# Autodesk Inventor assembly: GP4-100
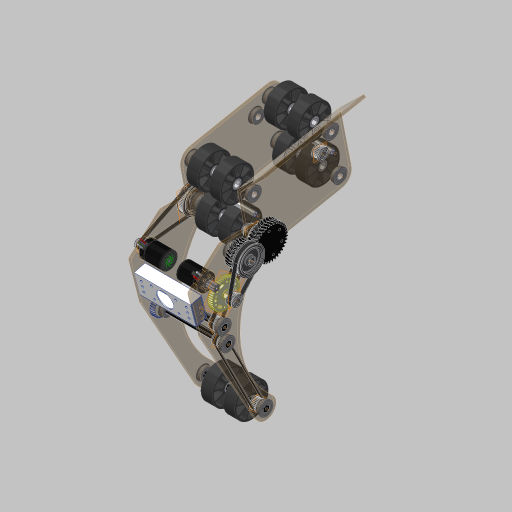
[picture p0: Inventor's stored thumbnail of the model, 512x512]
Saved by Autodesk Inventor 2023.5 (Build 275446000, 446)
## iProperties
Created: 2025-01-28
Part Number: GP4-100
Document SubType Name: Assembly
Designer: slick
Mass: 3583.72 g
Surface Area: 9499.92 cm^2
Volume: 1982.36 cm^3
Density: 1.80781 g/cm^3
Author: slick
## Documents named in this file (26)
- C:\Users\slick\OneDrive\Desktop\2025-ReefScape---CAD\Gripper\GP4\GP4-100.iam
- C:\Users\slick\OneDrive\Desktop\2025-ReefScape---CAD\Gripper\GP4\GP4-001.ipt
- C:\Users\slick\OneDrive\Desktop\2025-ReefScape---CAD\Gripper\GP4\GP4-002.ipt
- C:\Users\slick\OneDrive\Desktop\2025-ReefScape---CAD\Gripper\GP4\GP4-003.ipt
- C:\Users\slick\OneDrive\Desktop\2025-ReefScape---CAD\Gripper\GP4\GP4-003_MIR.ipt
- C:\Users\slick\OneDrive\Desktop\2025-ReefScape---CAD\COMMON PARTS\WHEELS\am-3945 3IN 500Hex Compliant Wheel REV 3.ipt
- C:\Users\slick\OneDrive\Desktop\2025-ReefScape---CAD\Gripper\GP4\GP4-005.ipt
- C:\Users\slick\OneDrive\Desktop\2025-ReefScape---CAD\Gripper\GP4\GP4-006.ipt
- C:\Users\slick\OneDrive\Desktop\2025-ReefScape---CAD\Gripper\GP4\GP4-007.ipt
- C:\Users\slick\OneDrive\Desktop\2025-ReefScape---CAD\COMMON PARTS\MOTORS\Minion.ipt
- C:\Users\slick\OneDrive\Desktop\2025-ReefScape---CAD\COMMON PARTS\PULLEYS\gt2\16T Gt2 Kracken PullyWCP-1178.ipt
- C:\Users\slick\OneDrive\Desktop\2025-ReefScape---CAD\COMMON PARTS\BEARINGS\13_75mm_1_2_ThunderHex_ID_x_1_125_OD_x_0_313_WD_Flanged_Bearing_217-4006_MIR.ipt
- C:\Users\slick\OneDrive\Desktop\2025-ReefScape---CAD\Gripper\GP4\GP4-008.ipt
- C:\Users\slick\OneDrive\Desktop\2025-ReefScape---CAD\COMMON PARTS\PULLEYS\gt2\60t_x_9mm_Wide_Double_Flange_Aluminum_Pulley_GT2_3mm_1_2_Hex_Bore_217-5876.ipt
- C:\Users\slick\OneDrive\Desktop\2025-ReefScape---CAD\COMMON PARTS\PULLEYS\gt2\24t_x_9mm_Wide_Double_Flange_Aluminum_Pulley_GT2_3mm_1_2_Hex_Bore_217-5875.ipt
- C:\Users\slick\OneDrive\Desktop\2025-ReefScape---CAD\COMMON PARTS\GEARS\20dp .5 hex\30t_Aluminum_Spur_Gear_20_DP_1_2_Hex_Bore_217-2705.ipt
- C:\Users\slick\OneDrive\Desktop\2025-ReefScape---CAD\Gripper\GP4\GP4-009.ipt
- C:\Users\slick\OneDrive\Desktop\2025-ReefScape---CAD\Gripper\GP4\GP4-010.ipt
- C:\Users\slick\OneDrive\Desktop\2025-ReefScape---CAD\COMMON PARTS\GEARS\Herringbone\herringbone 2m 24t\herringbone 2m 24t.ipt
- C:\Users\slick\OneDrive\Desktop\2025-ReefScape---CAD\COMMON PARTS\GEARS\Herringbone\2m 36t herringbone\2m 36t herringbone.ipt
- C:\Users\slick\OneDrive\Desktop\2025-ReefScape---CAD\COMMON PARTS\GEARS\WCP-1006\WCP-1006.ipt
- C:\Users\slick\OneDrive\Desktop\2025-ReefScape---CAD\COMMON PARTS\GEARS\20dp .5 hex\48t_Aluminum_Spur_Gear_20_DP_1_2_Hex_Bore_VersaKeys_217-3218.ipt
- C:\Users\slick\OneDrive\Desktop\2025-ReefScape---CAD\Gripper\GP4\90T GT2 Belt.ipt
- C:\Users\slick\OneDrive\Desktop\2025-ReefScape---CAD\Gripper\GP4\150T GT2 Belt.ipt
- C:\Users\slick\OneDrive\Desktop\2025-ReefScape---CAD\Gripper\GP4\130T GT2 Belt.ipt
- C:\Users\slick\OneDrive\Desktop\2025-ReefScape---CAD\Gripper\GP4\120T GT2 Belt.ipt
## Components (63 placed, 25 different names)
1. GP4-008:1 — Insert:1, Insert:2, Mate:2, Mate:6, Mate:11, Insert:21, Insert:26, Insert:27, Insert:28, Mate:41, Mate:42, Insert:29, Insert:30, Mate:49
2. GP4-002:1 — Flush:1, Flush:2, Flush:3, Mate:1, Flush:4, Flush:5
3. GP4-003:1 — Flush:1, Mate:1, Flush:4, Insert:1, Insert:2
4. GP4-003_MIR:1 — Flush:2, Flush:3, Flush:5, Insert:3, Insert:4
5. GP4-001:2 — Insert:3, Insert:4, Mate:7, Mate:10, Mate:12, Mate:23, Mate:24, Insert:7, Insert:14, Insert:15, Insert:16, Mate:27, Insert:19
6. GP4-006:1 — Mate:12, Mate:20, Mate:21, Mate:22, Symmetry:1, Insert:11, Insert:12, Insert:13, Mate:27, Insert:17, Insert:18, Insert:20, Insert:32, Mate:55
7. GP4-005:2 — Mate:11, Mate:15, Mate:22, Symmetry:1, Insert:5, Insert:6, Insert:22, Insert:23, Insert:24, Insert:25, Insert:33, Insert:34
8. GP4-007:1 — Insert:6, Insert:18
9. GP4-007:2 — Insert:5, Insert:17
10. Minion:1 — Mate:23, Mate:24, Insert:7, Mate:25, Flush:11, Mate:63
11. 16T Gt2 Kracken PullyWCP-1178:1 — Mate:25, Flush:11, Flush:29, Flush:30
12. 60t_x_9mm_Wide_Double_Flange_Aluminum_Pulley_GT2_3mm_1_2_Hex_Bore_217-5876:1 — Mate:28, Mate:54, Mate:61, Mate:64, Flush:30
13. 24t_x_9mm_Wide_Double_Flange_Aluminum_Pulley_GT2_3mm_1_2_Hex_Bore_217-5875:1 — Mate:32, Flush:14
14. 24t_x_9mm_Wide_Double_Flange_Aluminum_Pulley_GT2_3mm_1_2_Hex_Bore_217-5875:2 — Mate:31, Flush:13, Flush:14, Mate:62
15. 24t_x_9mm_Wide_Double_Flange_Aluminum_Pulley_GT2_3mm_1_2_Hex_Bore_217-5875:3 — Mate:30, Flush:13, Flush:17
16. 24t_x_9mm_Wide_Double_Flange_Aluminum_Pulley_GT2_3mm_1_2_Hex_Bore_217-5875:4 — Mate:29, Mate:37, Flush:17, Flush:28
17. 30t_Aluminum_Spur_Gear_20_DP_1_2_Hex_Bore_217-2705:1 — Mate:34, Flush:16, Mate:36, Mate:39, Flush:19
18. 30t_Aluminum_Spur_Gear_20_DP_1_2_Hex_Bore_217-2705:2 — Mate:35, Flush:16, Mate:38, Flush:18
19. GP4-009:1 — Mate:38, Flush:18
20. GP4-009:2 — Mate:39, Flush:19
21. GP4-010:1 — Mate:40, Flush:20
22. Minion:2 — Mate:41, Mate:42, Insert:29, Mate:48, Flush:23
23. herringbone 2m 24t:1 — Mate:44, Flush:22, Rotation:1, Mate:51, Mate:53
24. 24t_x_9mm_Wide_Double_Flange_Aluminum_Pulley_GT2_3mm_1_2_Hex_Bore_217-5875:5 — Mate:46, Flush:25
25. 24t_x_9mm_Wide_Double_Flange_Aluminum_Pulley_GT2_3mm_1_2_Hex_Bore_217-5875:6 — Mate:47
26. 2m 36t herringbone:1 — Insert:33, Insert:34, Flush:22, Rotation:1
27. WCP-1006:1 — Mate:48, Flush:23, Flush:26
28. 48t_Aluminum_Spur_Gear_20_DP_1_2_Hex_Bore_VersaKeys_217-3218:1 — Mate:49, Mate:50, Flush:26
29. 60t_x_9mm_Wide_Double_Flange_Aluminum_Pulley_GT2_3mm_1_2_Hex_Bore_217-5876:2 — Mate:51, Mate:53, Flush:24, Mate:57
30. 24t_x_9mm_Wide_Double_Flange_Aluminum_Pulley_GT2_3mm_1_2_Hex_Bore_217-5875:7 — Mate:50, Flush:24, Mate:56, Flush:27
31. 24t_x_9mm_Wide_Double_Flange_Aluminum_Pulley_GT2_3mm_1_2_Hex_Bore_217-5875:8 — Mate:54, Flush:25, Mate:55
32. 90T GT2 Belt:1 — Mate:56, Mate:57, Flush:27
33. 150T GT2 Belt:1 — Mate:58, Mate:59, Flush:28
34. 130T GT2 Belt:1 — Mate:60, Mate:61, Mate:62
35. 120T GT2 Belt:1 — Mate:63, Mate:64, Flush:29
36. am-3945 3IN 500Hex Compliant Wheel REV 3:10
37. am-3945 3IN 500Hex Compliant Wheel REV 3:9 — Mate:21, Flush:9
38. am-3945 3IN 500Hex Compliant Wheel REV 3:8
39. am-3945 3IN 500Hex Compliant Wheel REV 3:7 — Mate:20, Flush:10
40. am-3945 3IN 500Hex Compliant Wheel REV 3:6 — Mate:2, Mate:3, Flush:6, Flush:9
41. am-3945 3IN 500Hex Compliant Wheel REV 3:5 — Mate:3, Flush:7, Mate:10
42. am-3945 3IN 500Hex Compliant Wheel REV 3:4 — Mate:6, Mate:8
43. am-3945 3IN 500Hex Compliant Wheel REV 3:3 — Mate:7, Mate:8, Flush:8
44. am-3945 3IN 500Hex Compliant Wheel REV 3:2 — Mate:5, Mate:9, Flush:7, Flush:8
45. am-3945 3IN 500Hex Compliant Wheel REV 3:1 — Mate:5, Mate:9, Flush:6, Mate:15, Flush:10
46. 13_75mm_1_2_ThunderHex_ID_x_1_125_OD_x_0_313_WD_Flanged_Bearing_217-4006_MIR:19 — Insert:32, Mate:47
47. 13_75mm_1_2_ThunderHex_ID_x_1_125_OD_x_0_313_WD_Flanged_Bearing_217-4006_MIR:18 — Insert:30, Mate:44
48. 13_75mm_1_2_ThunderHex_ID_x_1_125_OD_x_0_313_WD_Flanged_Bearing_217-4006_MIR:10 — Insert:21
49. 13_75mm_1_2_ThunderHex_ID_x_1_125_OD_x_0_313_WD_Flanged_Bearing_217-4006_MIR:11 — Insert:22
50. 13_75mm_1_2_ThunderHex_ID_x_1_125_OD_x_0_313_WD_Flanged_Bearing_217-4006_MIR:12 — Insert:23
51. 13_75mm_1_2_ThunderHex_ID_x_1_125_OD_x_0_313_WD_Flanged_Bearing_217-4006_MIR:13 — Insert:24
52. 13_75mm_1_2_ThunderHex_ID_x_1_125_OD_x_0_313_WD_Flanged_Bearing_217-4006_MIR:14 — Insert:25
53. 13_75mm_1_2_ThunderHex_ID_x_1_125_OD_x_0_313_WD_Flanged_Bearing_217-4006_MIR:15 — Insert:28, Mate:60
54. 13_75mm_1_2_ThunderHex_ID_x_1_125_OD_x_0_313_WD_Flanged_Bearing_217-4006_MIR:16 — Insert:27, Mate:59
55. 13_75mm_1_2_ThunderHex_ID_x_1_125_OD_x_0_313_WD_Flanged_Bearing_217-4006_MIR:17 — Insert:26, Mate:37, Mate:58
56. 13_75mm_1_2_ThunderHex_ID_x_1_125_OD_x_0_313_WD_Flanged_Bearing_217-4006_MIR:1 — Insert:15, Mate:30, Mate:35
57. 13_75mm_1_2_ThunderHex_ID_x_1_125_OD_x_0_313_WD_Flanged_Bearing_217-4006_MIR:3 — Insert:20, Mate:32
58. 13_75mm_1_2_ThunderHex_ID_x_1_125_OD_x_0_313_WD_Flanged_Bearing_217-4006_MIR:4 — Insert:14, Mate:31, Mate:34, Mate:36
59. 13_75mm_1_2_ThunderHex_ID_x_1_125_OD_x_0_313_WD_Flanged_Bearing_217-4006_MIR:5 — Insert:13
60. 13_75mm_1_2_ThunderHex_ID_x_1_125_OD_x_0_313_WD_Flanged_Bearing_217-4006_MIR:6 — Insert:12
61. 13_75mm_1_2_ThunderHex_ID_x_1_125_OD_x_0_313_WD_Flanged_Bearing_217-4006_MIR:7 — Insert:11, Mate:46
62. 13_75mm_1_2_ThunderHex_ID_x_1_125_OD_x_0_313_WD_Flanged_Bearing_217-4006_MIR:8 — Insert:19, Mate:28
63. 13_75mm_1_2_ThunderHex_ID_x_1_125_OD_x_0_313_WD_Flanged_Bearing_217-4006_MIR:9 — Insert:16, Mate:29, Mate:40, Flush:20
## Relationships (115: Mate 56, Insert 30, Flush 27, Symmetry 1, RelateRotation 1)
- Flush:1: GP4-002:1 ↔ GP4-003:1
- Flush:2: GP4-002:1 ↔ GP4-003_MIR:1
- Flush:3: GP4-002:1 ↔ GP4-003_MIR:1
- Mate:1: GP4-002:1 ↔ GP4-003:1
- Flush:4: GP4-002:1 ↔ GP4-003:1
- Flush:5: GP4-002:1 ↔ GP4-003_MIR:1
- Insert:1: GP4-008:1 ↔ GP4-003:1
- Insert:2: GP4-008:1 ↔ GP4-003:1
- Insert:3: GP4-003_MIR:1 ↔ GP4-001:2
- Insert:4: GP4-003_MIR:1 ↔ GP4-001:2
- Mate:2: GP4-008:1 ↔ am-3945 3IN 500Hex Compliant Wheel REV 3:6
- Mate:3: am-3945 3IN 500Hex Compliant Wheel REV 3:6 ↔ am-3945 3IN 500Hex Compliant Wheel REV 3:5
- Mate:5: am-3945 3IN 500Hex Compliant Wheel REV 3:2 ↔ am-3945 3IN 500Hex Compliant Wheel REV 3:1
- Mate:6: GP4-008:1 ↔ am-3945 3IN 500Hex Compliant Wheel REV 3:4
- Mate:7: GP4-001:2 ↔ am-3945 3IN 500Hex Compliant Wheel REV 3:3
- Mate:8 (25.4 mm): am-3945 3IN 500Hex Compliant Wheel REV 3:4 ↔ am-3945 3IN 500Hex Compliant Wheel REV 3:3
- Mate:9 (25.4 mm): am-3945 3IN 500Hex Compliant Wheel REV 3:2 ↔ am-3945 3IN 500Hex Compliant Wheel REV 3:1
- Flush:6: am-3945 3IN 500Hex Compliant Wheel REV 3:6 ↔ am-3945 3IN 500Hex Compliant Wheel REV 3:1
- Flush:7: am-3945 3IN 500Hex Compliant Wheel REV 3:5 ↔ am-3945 3IN 500Hex Compliant Wheel REV 3:2
- Mate:10 (25.4 mm): GP4-001:2 ↔ am-3945 3IN 500Hex Compliant Wheel REV 3:5
- Flush:8: am-3945 3IN 500Hex Compliant Wheel REV 3:3 ↔ am-3945 3IN 500Hex Compliant Wheel REV 3:2
- Mate:11: GP4-008:1 ↔ GP4-005:2
- Mate:12: GP4-001:2 ↔ GP4-006:1
- Mate:15: GP4-005:2 ↔ am-3945 3IN 500Hex Compliant Wheel REV 3:1
- [Mate]: am-3945 3IN 500Hex Compliant Wheel REV 3:8 ↔ am-3945 3IN 500Hex Compliant Wheel REV 3:7
- [Mate] (25.4 mm): am-3945 3IN 500Hex Compliant Wheel REV 3:8 ↔ am-3945 3IN 500Hex Compliant Wheel REV 3:7
- [Mate]: am-3945 3IN 500Hex Compliant Wheel REV 3:10 ↔ am-3945 3IN 500Hex Compliant Wheel REV 3:9
- [Mate] (25.4 mm): am-3945 3IN 500Hex Compliant Wheel REV 3:10 ↔ am-3945 3IN 500Hex Compliant Wheel REV 3:9
- Mate:20: GP4-006:1 ↔ am-3945 3IN 500Hex Compliant Wheel REV 3:7
- Mate:21: GP4-006:1 ↔ am-3945 3IN 500Hex Compliant Wheel REV 3:9
- Flush:9: am-3945 3IN 500Hex Compliant Wheel REV 3:9 ↔ am-3945 3IN 500Hex Compliant Wheel REV 3:6
- Flush:10: am-3945 3IN 500Hex Compliant Wheel REV 3:7 ↔ am-3945 3IN 500Hex Compliant Wheel REV 3:1
- Mate:22: GP4-006:1 ↔ GP4-005:2
- Symmetry:1: GP4-006:1 ↔ GP4-005:2
- Insert:5: GP4-005:2 ↔ GP4-007:2
- Insert:6: GP4-005:2 ↔ GP4-007:1
- Mate:23: GP4-001:2 ↔ Minion:1
- Mate:24: GP4-001:2 ↔ Minion:1
- Insert:7: GP4-001:2 ↔ Minion:1
- Mate:25: Minion:1 ↔ 16T Gt2 Kracken PullyWCP-1178:1
- Flush:11: Minion:1 ↔ 16T Gt2 Kracken PullyWCP-1178:1
- Insert:11: GP4-006:1 ↔ 13_75mm_1_2_ThunderHex_ID_x_1_125_OD_x_0_313_WD_Flanged_Bearing_217-4006_MIR:7
- Insert:12: GP4-006:1 ↔ 13_75mm_1_2_ThunderHex_ID_x_1_125_OD_x_0_313_WD_Flanged_Bearing_217-4006_MIR:6
- Insert:13: GP4-006:1 ↔ 13_75mm_1_2_ThunderHex_ID_x_1_125_OD_x_0_313_WD_Flanged_Bearing_217-4006_MIR:5
- Insert:14: GP4-001:2 ↔ 13_75mm_1_2_ThunderHex_ID_x_1_125_OD_x_0_313_WD_Flanged_Bearing_217-4006_MIR:4
- Insert:15: GP4-001:2 ↔ 13_75mm_1_2_ThunderHex_ID_x_1_125_OD_x_0_313_WD_Flanged_Bearing_217-4006_MIR:1
- Insert:16: GP4-001:2 ↔ 13_75mm_1_2_ThunderHex_ID_x_1_125_OD_x_0_313_WD_Flanged_Bearing_217-4006_MIR:9
- Mate:27: GP4-001:2 ↔ GP4-006:1
- Insert:17: GP4-006:1 ↔ GP4-007:2
- Insert:18: GP4-006:1 ↔ GP4-007:1
- Insert:19: GP4-001:2 ↔ 13_75mm_1_2_ThunderHex_ID_x_1_125_OD_x_0_313_WD_Flanged_Bearing_217-4006_MIR:8
- Insert:20: GP4-006:1 ↔ 13_75mm_1_2_ThunderHex_ID_x_1_125_OD_x_0_313_WD_Flanged_Bearing_217-4006_MIR:3
- Mate:28: 60t_x_9mm_Wide_Double_Flange_Aluminum_Pulley_GT2_3mm_1_2_Hex_Bore_217-5876:1 ↔ 13_75mm_1_2_ThunderHex_ID_x_1_125_OD_x_0_313_WD_Flanged_Bearing_217-4006_MIR:8
- Mate:29: 24t_x_9mm_Wide_Double_Flange_Aluminum_Pulley_GT2_3mm_1_2_Hex_Bore_217-5875:4 ↔ 13_75mm_1_2_ThunderHex_ID_x_1_125_OD_x_0_313_WD_Flanged_Bearing_217-4006_MIR:9
- Mate:30: 24t_x_9mm_Wide_Double_Flange_Aluminum_Pulley_GT2_3mm_1_2_Hex_Bore_217-5875:3 ↔ 13_75mm_1_2_ThunderHex_ID_x_1_125_OD_x_0_313_WD_Flanged_Bearing_217-4006_MIR:1
- Mate:31: 24t_x_9mm_Wide_Double_Flange_Aluminum_Pulley_GT2_3mm_1_2_Hex_Bore_217-5875:2 ↔ 13_75mm_1_2_ThunderHex_ID_x_1_125_OD_x_0_313_WD_Flanged_Bearing_217-4006_MIR:4
- Mate:32: 24t_x_9mm_Wide_Double_Flange_Aluminum_Pulley_GT2_3mm_1_2_Hex_Bore_217-5875:1 ↔ 13_75mm_1_2_ThunderHex_ID_x_1_125_OD_x_0_313_WD_Flanged_Bearing_217-4006_MIR:3
- Flush:13: 24t_x_9mm_Wide_Double_Flange_Aluminum_Pulley_GT2_3mm_1_2_Hex_Bore_217-5875:2 ↔ 24t_x_9mm_Wide_Double_Flange_Aluminum_Pulley_GT2_3mm_1_2_Hex_Bore_217-5875:3
- Flush:14: 24t_x_9mm_Wide_Double_Flange_Aluminum_Pulley_GT2_3mm_1_2_Hex_Bore_217-5875:1 ↔ 24t_x_9mm_Wide_Double_Flange_Aluminum_Pulley_GT2_3mm_1_2_Hex_Bore_217-5875:2
- Mate:34: 30t_Aluminum_Spur_Gear_20_DP_1_2_Hex_Bore_217-2705:1 ↔ 13_75mm_1_2_ThunderHex_ID_x_1_125_OD_x_0_313_WD_Flanged_Bearing_217-4006_MIR:4
- Mate:35: 30t_Aluminum_Spur_Gear_20_DP_1_2_Hex_Bore_217-2705:2 ↔ 13_75mm_1_2_ThunderHex_ID_x_1_125_OD_x_0_313_WD_Flanged_Bearing_217-4006_MIR:1
- Flush:16: 30t_Aluminum_Spur_Gear_20_DP_1_2_Hex_Bore_217-2705:1 ↔ 30t_Aluminum_Spur_Gear_20_DP_1_2_Hex_Bore_217-2705:2
- Mate:36 (3.175 mm): 30t_Aluminum_Spur_Gear_20_DP_1_2_Hex_Bore_217-2705:1 ↔ 13_75mm_1_2_ThunderHex_ID_x_1_125_OD_x_0_313_WD_Flanged_Bearing_217-4006_MIR:4
- Insert:21: GP4-008:1 ↔ 13_75mm_1_2_ThunderHex_ID_x_1_125_OD_x_0_313_WD_Flanged_Bearing_217-4006_MIR:10
- Insert:22: GP4-005:2 ↔ 13_75mm_1_2_ThunderHex_ID_x_1_125_OD_x_0_313_WD_Flanged_Bearing_217-4006_MIR:11
- Insert:23: GP4-005:2 ↔ 13_75mm_1_2_ThunderHex_ID_x_1_125_OD_x_0_313_WD_Flanged_Bearing_217-4006_MIR:12
- Insert:24: GP4-005:2 ↔ 13_75mm_1_2_ThunderHex_ID_x_1_125_OD_x_0_313_WD_Flanged_Bearing_217-4006_MIR:13
- Insert:25: GP4-005:2 ↔ 13_75mm_1_2_ThunderHex_ID_x_1_125_OD_x_0_313_WD_Flanged_Bearing_217-4006_MIR:14
- Insert:26: GP4-008:1 ↔ 13_75mm_1_2_ThunderHex_ID_x_1_125_OD_x_0_313_WD_Flanged_Bearing_217-4006_MIR:17
- Insert:27: GP4-008:1 ↔ 13_75mm_1_2_ThunderHex_ID_x_1_125_OD_x_0_313_WD_Flanged_Bearing_217-4006_MIR:16
- Insert:28: GP4-008:1 ↔ 13_75mm_1_2_ThunderHex_ID_x_1_125_OD_x_0_313_WD_Flanged_Bearing_217-4006_MIR:15
- Mate:37 (3.175 mm): 24t_x_9mm_Wide_Double_Flange_Aluminum_Pulley_GT2_3mm_1_2_Hex_Bore_217-5875:4 ↔ 13_75mm_1_2_ThunderHex_ID_x_1_125_OD_x_0_313_WD_Flanged_Bearing_217-4006_MIR:17
- Flush:17: 24t_x_9mm_Wide_Double_Flange_Aluminum_Pulley_GT2_3mm_1_2_Hex_Bore_217-5875:3 ↔ 24t_x_9mm_Wide_Double_Flange_Aluminum_Pulley_GT2_3mm_1_2_Hex_Bore_217-5875:4
- Mate:38: 30t_Aluminum_Spur_Gear_20_DP_1_2_Hex_Bore_217-2705:2 ↔ GP4-009:1
- Mate:39: 30t_Aluminum_Spur_Gear_20_DP_1_2_Hex_Bore_217-2705:1 ↔ GP4-009:2
- Flush:18: 30t_Aluminum_Spur_Gear_20_DP_1_2_Hex_Bore_217-2705:2 ↔ GP4-009:1
- Flush:19: 30t_Aluminum_Spur_Gear_20_DP_1_2_Hex_Bore_217-2705:1 ↔ GP4-009:2
- Mate:40: GP4-010:1 ↔ 13_75mm_1_2_ThunderHex_ID_x_1_125_OD_x_0_313_WD_Flanged_Bearing_217-4006_MIR:9
- Flush:20: GP4-010:1 ↔ 13_75mm_1_2_ThunderHex_ID_x_1_125_OD_x_0_313_WD_Flanged_Bearing_217-4006_MIR:9
- Mate:41: GP4-008:1 ↔ Minion:2
- Mate:42: GP4-008:1 ↔ Minion:2
- Insert:29: GP4-008:1 ↔ Minion:2
- Insert:30: GP4-008:1 ↔ 13_75mm_1_2_ThunderHex_ID_x_1_125_OD_x_0_313_WD_Flanged_Bearing_217-4006_MIR:18
- Mate:44: herringbone 2m 24t:1 ↔ 13_75mm_1_2_ThunderHex_ID_x_1_125_OD_x_0_313_WD_Flanged_Bearing_217-4006_MIR:18
- Insert:32: GP4-006:1 ↔ 13_75mm_1_2_ThunderHex_ID_x_1_125_OD_x_0_313_WD_Flanged_Bearing_217-4006_MIR:19
- Mate:46: 24t_x_9mm_Wide_Double_Flange_Aluminum_Pulley_GT2_3mm_1_2_Hex_Bore_217-5875:5 ↔ 13_75mm_1_2_ThunderHex_ID_x_1_125_OD_x_0_313_WD_Flanged_Bearing_217-4006_MIR:7
- Mate:47: 24t_x_9mm_Wide_Double_Flange_Aluminum_Pulley_GT2_3mm_1_2_Hex_Bore_217-5875:6 ↔ 13_75mm_1_2_ThunderHex_ID_x_1_125_OD_x_0_313_WD_Flanged_Bearing_217-4006_MIR:19
- Insert:33: GP4-005:2 ↔ 2m 36t herringbone:1
- Insert:34: GP4-005:2 ↔ 2m 36t herringbone:1
- Flush:22: herringbone 2m 24t:1 ↔ 2m 36t herringbone:1
- Rotation:1 [RelateRotation] (1 ul): herringbone 2m 24t:1 ↔ 2m 36t herringbone:1
- Mate:48: Minion:2 ↔ WCP-1006:1
- Flush:23: Minion:2 ↔ WCP-1006:1
- Mate:49: GP4-008:1 ↔ 48t_Aluminum_Spur_Gear_20_DP_1_2_Hex_Bore_VersaKeys_217-3218:1
- Mate:50: 48t_Aluminum_Spur_Gear_20_DP_1_2_Hex_Bore_VersaKeys_217-3218:1 ↔ 24t_x_9mm_Wide_Double_Flange_Aluminum_Pulley_GT2_3mm_1_2_Hex_Bore_217-5875:7
- Mate:51: herringbone 2m 24t:1 ↔ 60t_x_9mm_Wide_Double_Flange_Aluminum_Pulley_GT2_3mm_1_2_Hex_Bore_217-5876:2
- Mate:53: herringbone 2m 24t:1 ↔ 60t_x_9mm_Wide_Double_Flange_Aluminum_Pulley_GT2_3mm_1_2_Hex_Bore_217-5876:2
- Flush:24: 60t_x_9mm_Wide_Double_Flange_Aluminum_Pulley_GT2_3mm_1_2_Hex_Bore_217-5876:2 ↔ 24t_x_9mm_Wide_Double_Flange_Aluminum_Pulley_GT2_3mm_1_2_Hex_Bore_217-5875:7
- Mate:54: 60t_x_9mm_Wide_Double_Flange_Aluminum_Pulley_GT2_3mm_1_2_Hex_Bore_217-5876:1 ↔ 24t_x_9mm_Wide_Double_Flange_Aluminum_Pulley_GT2_3mm_1_2_Hex_Bore_217-5875:8
- Flush:25: 24t_x_9mm_Wide_Double_Flange_Aluminum_Pulley_GT2_3mm_1_2_Hex_Bore_217-5875:5 ↔ 24t_x_9mm_Wide_Double_Flange_Aluminum_Pulley_GT2_3mm_1_2_Hex_Bore_217-5875:8
- Mate:55 (1.5875 mm): GP4-006:1 ↔ 24t_x_9mm_Wide_Double_Flange_Aluminum_Pulley_GT2_3mm_1_2_Hex_Bore_217-5875:8
- Flush:26: WCP-1006:1 ↔ 48t_Aluminum_Spur_Gear_20_DP_1_2_Hex_Bore_VersaKeys_217-3218:1
- Mate:56: 24t_x_9mm_Wide_Double_Flange_Aluminum_Pulley_GT2_3mm_1_2_Hex_Bore_217-5875:7 ↔ 90T GT2 Belt:1
- Mate:57 (0.0762 mm): 60t_x_9mm_Wide_Double_Flange_Aluminum_Pulley_GT2_3mm_1_2_Hex_Bore_217-5876:2 ↔ 90T GT2 Belt:1
- Flush:27: 24t_x_9mm_Wide_Double_Flange_Aluminum_Pulley_GT2_3mm_1_2_Hex_Bore_217-5875:7 ↔ 90T GT2 Belt:1
- Mate:58: 150T GT2 Belt:1 ↔ 13_75mm_1_2_ThunderHex_ID_x_1_125_OD_x_0_313_WD_Flanged_Bearing_217-4006_MIR:17
- Mate:59: 150T GT2 Belt:1 ↔ 13_75mm_1_2_ThunderHex_ID_x_1_125_OD_x_0_313_WD_Flanged_Bearing_217-4006_MIR:16
- Flush:28: 24t_x_9mm_Wide_Double_Flange_Aluminum_Pulley_GT2_3mm_1_2_Hex_Bore_217-5875:4 ↔ 150T GT2 Belt:1
- Mate:60: 130T GT2 Belt:1 ↔ 13_75mm_1_2_ThunderHex_ID_x_1_125_OD_x_0_313_WD_Flanged_Bearing_217-4006_MIR:15
- Mate:61: 60t_x_9mm_Wide_Double_Flange_Aluminum_Pulley_GT2_3mm_1_2_Hex_Bore_217-5876:1 ↔ 130T GT2 Belt:1
- Mate:62: 24t_x_9mm_Wide_Double_Flange_Aluminum_Pulley_GT2_3mm_1_2_Hex_Bore_217-5875:2 ↔ 130T GT2 Belt:1
- Mate:63: Minion:1 ↔ 120T GT2 Belt:1
- Mate:64 (0.0762 mm): 60t_x_9mm_Wide_Double_Flange_Aluminum_Pulley_GT2_3mm_1_2_Hex_Bore_217-5876:1 ↔ 120T GT2 Belt:1
- Flush:29: 16T Gt2 Kracken PullyWCP-1178:1 ↔ 120T GT2 Belt:1
- Flush:30: 16T Gt2 Kracken PullyWCP-1178:1 ↔ 60t_x_9mm_Wide_Double_Flange_Aluminum_Pulley_GT2_3mm_1_2_Hex_Bore_217-5876:1
## Named parameters: d53_d33 = 0 mm, d54_d37 = 25.4 mm, d55_d33 = 0 mm, d56_d37 = 25.4 mm
